# Autodesk Inventor assembly: fan_unit_01
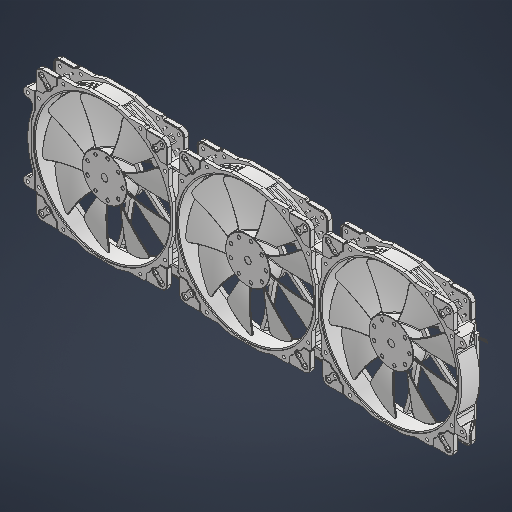
[picture p0: Inventor's stored thumbnail of the model, 512x512]
Saved by Autodesk Inventor 2026.2 (Build 302298010, 298A)
## iProperties
Created: 2026-05-14
Part Number: fan_unit_01
Document SubType Name: Assembly
Designer: nyxeon
Author: nyxeon
## Documents named in this file (4)
- C:\Users\nyxeon\Documents\CAD\Inventor\eatx_case\robocup\fan_unit_01.iam
- C:\Users\nyxeon\Documents\CAD\Inventor\eatx_case\robocup\parts\fan_noctua_nf-a20_assembly\fan_noctua_nf-a20_assembly\fan_noctua_nf-a20_assembly.iam
- C:\Users\nyxeon\Documents\CAD\Inventor\eatx_case\robocup\fan_connector_01.ipt
- C:\Users\nyxeon\Documents\CAD\Inventor\eatx_case\robocup\fan_connector_02.ipt
## Components (7 placed, 3 different names)
1. fan_noctua_nf-a20_assembly:1 [sub-assembly] — フラッシュ:1, フラッシュ:2, フラッシュ:3, フラッシュ:4, メイト:1, メイト:2, メイト:3
2. fan_noctua_nf-a20_assembly:2 [sub-assembly] — フラッシュ:2, フラッシュ:3, メイト:1, メイト:4, メイト:7, メイト:8
3. fan_noctua_nf-a20_assembly:3 [sub-assembly] — フラッシュ:1, フラッシュ:4, メイト:2, メイト:5, メイト:6
4. fan_connector_01:1 — フラッシュ:5, フラッシュ:6, フラッシュ:7
5. fan_connector_01:2 — フラッシュ:6, メイト:3, メイト:4
6. fan_connector_02:1 — メイト:7, メイト:8, フラッシュ:8
7. fan_connector_02:2 — メイト:5, メイト:6, フラッシュ:7, フラッシュ:8
## Relationships (16: Flush 8, Mate 8)
- フラッシュ:1 [Flush]: fan_noctua_nf-a20_assembly:1 ↔ fan_noctua_nf-a20_assembly:3
- フラッシュ:2 [Flush]: fan_noctua_nf-a20_assembly:1 ↔ fan_noctua_nf-a20_assembly:2
- フラッシュ:3 [Flush]: fan_noctua_nf-a20_assembly:1 ↔ fan_noctua_nf-a20_assembly:2
- フラッシュ:4 [Flush]: fan_noctua_nf-a20_assembly:1 ↔ fan_noctua_nf-a20_assembly:3
- メイト:1 [Mate] (4.25 mm): fan_noctua_nf-a20_assembly:1 ↔ fan_noctua_nf-a20_assembly:2
- メイト:2 [Mate] (4.25 mm): fan_noctua_nf-a20_assembly:1 ↔ fan_noctua_nf-a20_assembly:3
- フラッシュ:5 [Flush]: fan_connector_01:1
- フラッシュ:6 [Flush]: fan_connector_01:1 ↔ fan_connector_01:2
- メイト:3 [Mate]: fan_noctua_nf-a20_assembly:1 ↔ fan_connector_01:2
- メイト:4 [Mate]: fan_noctua_nf-a20_assembly:2 ↔ fan_connector_01:2
- メイト:5 [Mate]: fan_noctua_nf-a20_assembly:3 ↔ fan_connector_02:2
- メイト:6 [Mate]: fan_noctua_nf-a20_assembly:3 ↔ fan_connector_02:2
- フラッシュ:7 [Flush]: fan_connector_01:1 ↔ fan_connector_02:2
- メイト:7 [Mate]: fan_noctua_nf-a20_assembly:2 ↔ fan_connector_02:1
- メイト:8 [Mate]: fan_noctua_nf-a20_assembly:2 ↔ fan_connector_02:1
- フラッシュ:8 [Flush]: fan_connector_02:1 ↔ fan_connector_02:2
